# Autodesk Inventor assembly: SSEB6L-145-B3
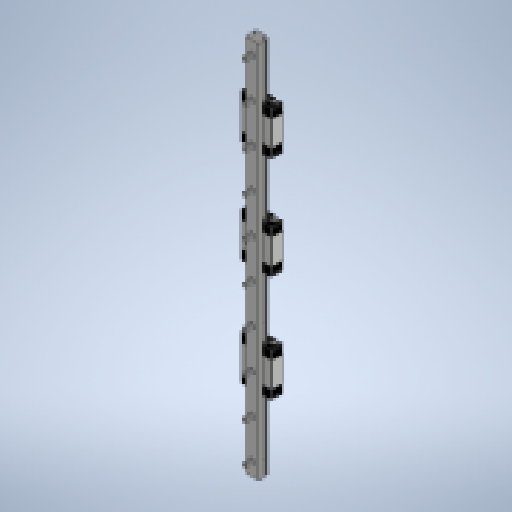
[picture p0: Inventor's stored thumbnail of the model, 512x512]
Saved by Autodesk Inventor 2024.3 (Build 283343000, 343)
## iProperties
Category: PARTsolutions
Company: MISUMI
Created: 2025-06-10
Part Number: SSEB6L-145-B3
Catalog Web Link: www.cadenas.de
Description: SSEB, SSEB-MX, SSE2B, SSE2B-MX, RSEB, RSE2B-Miniature Linear Guides Standard Blocks/Light Preload High Grade-L Selectable Type
Vendor: MISUMI
Document SubType Name: Assembly
Designer: psAdmin
Manufacturer: MISUMI
Mass: 4.72625 g
Surface Area: 62.8067 cm^2
Volume: 4.72625 cm^3
PSOL_IDENT_0: {$CADENAS_DATA/23d-libs/misumi/metric/06_linear_guides/re2b_asmtab.prj},262 {VTYP=3D},{STYP=ASSTAB},
PSOL_IDENT_1: {NB=SSEB6L-145-B3},{LINA=SSEB6L-145-B3},{NN=SSEB, SSEB-MX, SSE2B, SSE2B-MX, RSEB, RSE2B},{DATE=04.04
PSOL_IDENT_2: .2024 07:12:35},{GEOMDATE=07.03.2024 00:33:43},{VERSION=},{LINEID=60},{WBVAR=ST,MAT,MX,NOB,GREASE,LS
PSOL_IDENT_3: ,ALT1,ALT2,ALT3,ALT4},{WBNUMERIC=LS}  {NB=SSEB6L-145-B3},{LINA=SSEB6L-145-B3},{KT=DUMMY},{PN=SSEB6L-
PSOL_IDENT_4: 145-B3},{RT=B},{TYPE=SSEB},{ST=S},{MAT=S},{MX=},{MXALG= '','w/o MX(Lubrication unit)' },{NOB=},{H=6}
PSOL_IDENT_5: ,{GREASE=L},{GREASEALG='','Normal', 'L'  , 'L Type Greased ', 'G', 'G Type Greased', 'Y', 'Y Type Gr
PSOL_IDENT_6: eased', 'H', 'H Type Greased'},{LT=Selectable},{LS=145},{HARD=56HRC~},{W=12},{L1=17.4},{B=8},{C=0},{
PSOL_IDENT_7: SLL=M2x1.5},{L2=9.7},{K=4.5},{CBB=0.3},{W1=5},{W2=3.5},{H1=4.0},{CAA=0.3},{DD1DD2HH=2.4x3.5x1},{F=15
PSOL_IDENT_8: },{G=5.0},{ALT1=},{ALT1ALG= '', 'w/o MC (Tapped Holes)' },{MC=M2.6},{ALT2=},{ALT2L=0.0},{ALT2N=0},{M=
PSOL_IDENT_9: 10},{LL=},{L0=25,40,55,70,85,100,115,130,145},{REC1=   '','Not applicable'    },{ST1='S', 'w/o Surfa
PSOL_IDENT_10: ce Treatment'},{MAT2='S','Stainless Steel'},{ALT3=},{ALT3ALG= '' , 'w/o WC (Pair of Rails)' , '-WC'
PSOL_IDENT_11: , 'with WC (Set Pair of Rails)' },{ALT4=-B3},{ALT4ALG= '','w/o (Additional Blocks)','-B3','with B3(3
PSOL_IDENT_12: -Block Type (Adds 2 blocks.))' },{PPATH=seb_series/seb_asmtpl.prj}
NB: SSEB6L-145-B3
NN: SSEB, SSEB-MX, SSE2B, SSE2B-MX, RSEB, RSE2B
NT: Miniature Linear Guides Standard Blocks/Light Preload High Grade-L Selectable Type
NBSYN: $PN.
LINA: SSEB6L-145-B3
CATALOG: Misumi
PN: SSEB6L-145-B3
ST: w/o Surface Treatment
MAT: Stainless Steel
MX: w/o MX(Lubrication unit)
NOB: 1
H: 6
GREASE: L Type Greased
LS: 145
W: 12
L1: 17.4
B: 8
C: 0
SLL: M2x1.5
L2: 9.7
K: 4.5
CBB: 0.3
W1: 5
W2: 3.5
H1: 4
CAA: 0.3
DD1DD2HH: 2.4x3.5x1
F: 15
G: 5
ALT1: w/o MC (Tapped Holes)
ALT2: Not applicable
ALT3: w/o WC (Pair of Rails)
ALT4: with B3(3-Block Type (Adds 2 blocks.))
SUPPLIER: MISUMI
ARTICLENO: SSEB6L-145-B3
BOMINFO: SSEB6L-145-B3
CREATOR: CADENAS GmbH
Title: SSEB6L-145-B3
Author: Cadenas PARTsolutions
Comments: Miniature Linear Guides Standard Blocks/Light Preload High Grade-L Selectable Type
## Documents named in this file (4)
- C:\Users\hikou\OneDrive\ドキュメント\Inventor\end_effector\harvesting_endeffector\linear_slider\AIS2024\SSEB6L-145-B3.iam
- C:\Users\hikou\OneDrive\ドキュメント\Inventor\end_effector\harvesting_endeffector\linear_slider\AIS2024\SSEB6-145-B3_r.ipt
- C:\Users\hikou\OneDrive\ドキュメント\Inventor\end_effector\harvesting_endeffector\linear_slider\AIS2024\SSEB6_b.ipt
- C:\Users\hikou\OneDrive\ドキュメント\Inventor\end_effector\harvesting_endeffector\linear_slider\AIS2024\M2x6_b.ipt
## Components (14 placed, 3 different names)
1. SSEB6-145-B3_r:1 — to_block_Z@1 <-> to_rail_Z@2, to_block_YZ@1 <-> to_rail_YZ@2, to_block_2_Z@1 <-> to_rail_Z@3, to_block_2_YZ@1 <-> to_rail_YZ@3, to_block_3_Z@1 <-> to_rail_Z@4, to_block_3_YZ@1 <-> to_rail_YZ@4, screw_1_Z@1 <-> screw_to_rail_Z@5, screw_1_YZ@1 <-> screw_to_rail_YZ@5, screw_2_Z@1 <-> screw_to_rail_Z@6, screw_2_YZ@1 <-> screw_to_rail_YZ@6, screw_3_Z@1 <-> screw_to_rail_Z@7, screw_3_YZ@1 <-> screw_to_rail_YZ@7, screw_4_Z@1 <-> screw_to_rail_Z@8, screw_4_YZ@1 <-> screw_to_rail_YZ@8, screw_5_Z@1 <-> screw_to_rail_Z@9, screw_5_YZ@1 <-> screw_to_rail_YZ@9, screw_6_Z@1 <-> screw_to_rail_Z@10, screw_6_YZ@1 <-> screw_to_rail_YZ@10, screw_7_Z@1 <-> screw_to_rail_Z@11, screw_7_YZ@1 <-> screw_to_rail_YZ@11, screw_8_Z@1 <-> screw_to_rail_Z@12, screw_8_YZ@1 <-> screw_to_rail_YZ@12, screw_9_Z@1 <-> screw_to_rail_Z@13, screw_9_YZ@1 <-> screw_to_rail_YZ@13, screw_10_Z@1 <-> screw_to_rail_Z@14, screw_10_YZ@1 <-> screw_to_rail_YZ@14
2. SSEB6_b:1 — to_block_Z@1 <-> to_rail_Z@2, to_block_YZ@1 <-> to_rail_YZ@2
3. SSEB6_b:2 — to_block_2_Z@1 <-> to_rail_Z@3, to_block_2_YZ@1 <-> to_rail_YZ@3
4. SSEB6_b:3 — to_block_3_Z@1 <-> to_rail_Z@4, to_block_3_YZ@1 <-> to_rail_YZ@4
5. M2x6_b:1 — screw_1_Z@1 <-> screw_to_rail_Z@5, screw_1_YZ@1 <-> screw_to_rail_YZ@5
6. M2x6_b:2 — screw_2_Z@1 <-> screw_to_rail_Z@6, screw_2_YZ@1 <-> screw_to_rail_YZ@6
7. M2x6_b:3 — screw_3_Z@1 <-> screw_to_rail_Z@7, screw_3_YZ@1 <-> screw_to_rail_YZ@7
8. M2x6_b:4 — screw_4_Z@1 <-> screw_to_rail_Z@8, screw_4_YZ@1 <-> screw_to_rail_YZ@8
9. M2x6_b:5 — screw_5_Z@1 <-> screw_to_rail_Z@9, screw_5_YZ@1 <-> screw_to_rail_YZ@9
10. M2x6_b:6 — screw_6_Z@1 <-> screw_to_rail_Z@10, screw_6_YZ@1 <-> screw_to_rail_YZ@10
11. M2x6_b:7 — screw_7_Z@1 <-> screw_to_rail_Z@11, screw_7_YZ@1 <-> screw_to_rail_YZ@11
12. M2x6_b:8 — screw_8_Z@1 <-> screw_to_rail_Z@12, screw_8_YZ@1 <-> screw_to_rail_YZ@12
13. M2x6_b:9 — screw_9_Z@1 <-> screw_to_rail_Z@13, screw_9_YZ@1 <-> screw_to_rail_YZ@13
14. M2x6_b:10 — screw_10_Z@1 <-> screw_to_rail_Z@14, screw_10_YZ@1 <-> screw_to_rail_YZ@14
## Relationships (26: Mate 13, Angle 13)
- to_block_Z@1 <-> to_rail_Z@2 [Mate]: SSEB6-145-B3_r:1 ↔ SSEB6_b:1
- to_block_YZ@1 <-> to_rail_YZ@2 [Angle] (0 deg): SSEB6-145-B3_r:1 ↔ SSEB6_b:1
- to_block_2_Z@1 <-> to_rail_Z@3 [Mate]: SSEB6-145-B3_r:1 ↔ SSEB6_b:2
- to_block_2_YZ@1 <-> to_rail_YZ@3 [Angle] (0 deg): SSEB6-145-B3_r:1 ↔ SSEB6_b:2
- to_block_3_Z@1 <-> to_rail_Z@4 [Mate]: SSEB6-145-B3_r:1 ↔ SSEB6_b:3
- to_block_3_YZ@1 <-> to_rail_YZ@4 [Angle] (0 deg): SSEB6-145-B3_r:1 ↔ SSEB6_b:3
- screw_1_Z@1 <-> screw_to_rail_Z@5 [Mate]: SSEB6-145-B3_r:1 ↔ M2x6_b:1
- screw_1_YZ@1 <-> screw_to_rail_YZ@5 [Angle] (0 deg): SSEB6-145-B3_r:1 ↔ M2x6_b:1
- screw_2_Z@1 <-> screw_to_rail_Z@6 [Mate]: SSEB6-145-B3_r:1 ↔ M2x6_b:2
- screw_2_YZ@1 <-> screw_to_rail_YZ@6 [Angle] (0 deg): SSEB6-145-B3_r:1 ↔ M2x6_b:2
- screw_3_Z@1 <-> screw_to_rail_Z@7 [Mate]: SSEB6-145-B3_r:1 ↔ M2x6_b:3
- screw_3_YZ@1 <-> screw_to_rail_YZ@7 [Angle] (0 deg): SSEB6-145-B3_r:1 ↔ M2x6_b:3
- screw_4_Z@1 <-> screw_to_rail_Z@8 [Mate]: SSEB6-145-B3_r:1 ↔ M2x6_b:4
- screw_4_YZ@1 <-> screw_to_rail_YZ@8 [Angle] (0 deg): SSEB6-145-B3_r:1 ↔ M2x6_b:4
- screw_5_Z@1 <-> screw_to_rail_Z@9 [Mate]: SSEB6-145-B3_r:1 ↔ M2x6_b:5
- screw_5_YZ@1 <-> screw_to_rail_YZ@9 [Angle] (0 deg): SSEB6-145-B3_r:1 ↔ M2x6_b:5
- screw_6_Z@1 <-> screw_to_rail_Z@10 [Mate]: SSEB6-145-B3_r:1 ↔ M2x6_b:6
- screw_6_YZ@1 <-> screw_to_rail_YZ@10 [Angle] (0 deg): SSEB6-145-B3_r:1 ↔ M2x6_b:6
- screw_7_Z@1 <-> screw_to_rail_Z@11 [Mate]: SSEB6-145-B3_r:1 ↔ M2x6_b:7
- screw_7_YZ@1 <-> screw_to_rail_YZ@11 [Angle] (0 deg): SSEB6-145-B3_r:1 ↔ M2x6_b:7
- screw_8_Z@1 <-> screw_to_rail_Z@12 [Mate]: SSEB6-145-B3_r:1 ↔ M2x6_b:8
- screw_8_YZ@1 <-> screw_to_rail_YZ@12 [Angle] (0 deg): SSEB6-145-B3_r:1 ↔ M2x6_b:8
- screw_9_Z@1 <-> screw_to_rail_Z@13 [Mate]: SSEB6-145-B3_r:1 ↔ M2x6_b:9
- screw_9_YZ@1 <-> screw_to_rail_YZ@13 [Angle] (0 deg): SSEB6-145-B3_r:1 ↔ M2x6_b:9
- screw_10_Z@1 <-> screw_to_rail_Z@14 [Mate]: SSEB6-145-B3_r:1 ↔ M2x6_b:10
- screw_10_YZ@1 <-> screw_to_rail_YZ@14 [Angle] (0 deg): SSEB6-145-B3_r:1 ↔ M2x6_b:10
